# Autodesk Inventor assembly: V2 modular session template
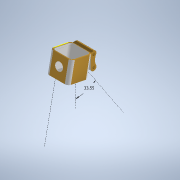
[picture p0: Inventor's stored thumbnail of the model, 180x180]
Saved by Autodesk Inventor 2020 (Build 240168000, 168)
## iProperties
Created: 2022-08-01
Part Number: V2 modular session template
Document SubType Name: Assembly
Designer: Steven
Author: Steven
## Documents named in this file (3)
- Y:\FPV drone stuff\0 Street League\Frames\PB-Kauri-X\3D prints\35 mm canopy\work in progress prints\session mounts\V2 modular session template.iam
- Y:\FPV drone stuff\0 Street League\Frames\PB-Kauri-X\3D prints\35 mm canopy\work in progress prints\session mounts\V2 modular session camera case.ipt
- Y:\FPV drone stuff\0 Street League\Frames\PB-Kauri-X\3D prints\35 mm canopy\work in progress prints\session mounts\V2 modular session frame mount.ipt
## Components (2 placed, 2 different names)
1. V2 modular session camera case:1 — Flush:4, Mate:1, Angle:1
2. V2 modular session frame mount:1 — Flush:1, Flush:2, Flush:3, Flush:4, Mate:1, Angle:1
## Relationships (6: Flush 4, Mate 1, Angle 1)
- Flush:1: V2 modular session frame mount:1
- Flush:2: V2 modular session frame mount:1
- Flush:3: V2 modular session frame mount:1
- Flush:4: V2 modular session camera case:1 ↔ V2 modular session frame mount:1
- Mate:1: V2 modular session camera case:1 ↔ V2 modular session frame mount:1
- Angle:1 (45 deg): V2 modular session camera case:1 ↔ V2 modular session frame mount:1
